# Autodesk Inventor assembly: Assembly146-01
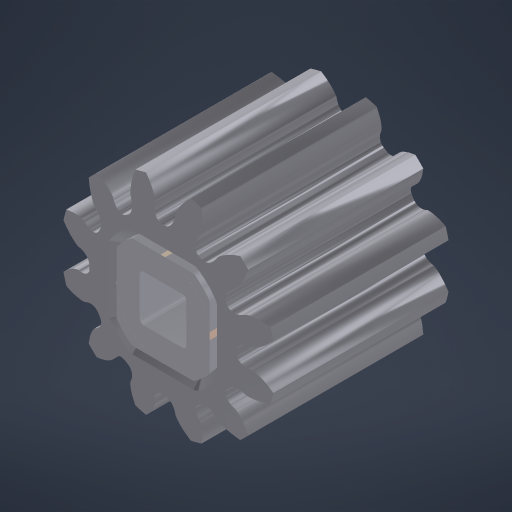
[picture p0: Inventor's stored thumbnail of the model, 512x512]
Saved by Autodesk Inventor 2024 (Build 280153000, 153)
## iProperties
Created: 2022-08-02
Part Number: Assembly146-01
Document SubType Name: Assembly
Designer: ylu12
Author: ylu12
## Documents named in this file (4)
- \\Mac\Home\Desktop\code\1599V-VRC\Cad\Motion\Gears\HS Gear\HS 12T Gear, Square.iam
- \\Mac\Home\Desktop\code\1599V-VRC\Cad\Motion\HS Shaft Adapter Square.ipt
- \\Mac\Home\Desktop\code\1599V-VRC\Cad\Motion\Gears\Reference Files\HS 12T Gear, No Insert.ipt
- \\Mac\Home\Desktop\code\1599V-VRC\Cad\Motion\Gears\HS Gear.iam
## Components (2 placed, 2 different names)
1. Square — Mate:3, Mate:4, Flush:2
2. 12T — Mate:5, Mate:6, Flush:3
## Relationships (6: Mate 4, Flush 2)
- Mate:3: Square
- Mate:4: Square
- Flush:2 (6.35 mm): Square
- Mate:5: 12T
- Mate:6: 12T
- Flush:3: 12T
